# Autodesk Inventor assembly: mezzanineBoard2
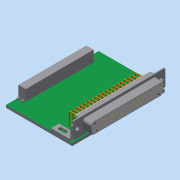
[picture p0: Inventor's stored thumbnail of the model, 180x180]
Saved by Autodesk Inventor 2016 (Build 200138000, 138)
## iProperties
Created: 2016-08-31
Part Number: mezzanineBoard2
Document SubType Name: Assembly
Designer: Zara
Author: Zara
## Documents named in this file (5)
- C:\Users\Zara\Documents\hera-cad\Node\SNAP V2 enclosure release - pack-n-go export\SNAP V2 enclosure release - pack-n-go export\Workspaces\Workspace\components\mezzanineBoard2.iam
- C:\Users\Zara\Documents\hera-cad\Node\SNAP V2 enclosure release - pack-n-go export\SNAP V2 enclosure release - pack-n-go export\Workspaces\Workspace\components\mezzaninePCB.ipt
- C:\Users\Zara\Documents\hera-cad\Node\SNAP V2 enclosure release - pack-n-go export\SNAP V2 enclosure release - pack-n-go export\Workspaces\Workspace\components\snapPinout.ipt
- C:\Users\Zara\Documents\hera-cad\Node\SNAP V2 enclosure release - pack-n-go export\SNAP V2 enclosure release - pack-n-go export\Workspaces\Workspace\components\dsub37Bracket.ipt
- C:\Users\Zara\Documents\hera-cad\Node\SNAP V2 enclosure release - pack-n-go export\SNAP V2 enclosure release - pack-n-go export\Workspaces\Workspace\components\174E-037-213.ipt
## Components (5 placed, 4 different names)
1. mezzaninePCB:1 — Mate:2, Flush:3, Flush:4, Mate:5, Mate:8, Flush:6, Flush:9, Flush:10
2. snapPinout:1 — Mate:2, Flush:3, Flush:4
3. dsub37Bracket:1 — Mate:5, Flush:9, Mate:9
4. dsub37Bracket:2 — Mate:8, Flush:6, Mate:10, Mate:11
5. 174E-037-213:1 — Mate:9, Mate:10, Flush:10, Mate:11
## Relationships (11: Mate 6, Flush 5)
- Mate:2: mezzaninePCB:1 ↔ snapPinout:1
- Flush:3: mezzaninePCB:1 ↔ snapPinout:1
- Flush:4 (9.3 mm): mezzaninePCB:1 ↔ snapPinout:1
- Mate:5: mezzaninePCB:1 ↔ dsub37Bracket:1
- Mate:8: mezzaninePCB:1 ↔ dsub37Bracket:2
- Flush:6: mezzaninePCB:1 ↔ dsub37Bracket:2
- Flush:9: mezzaninePCB:1 ↔ dsub37Bracket:1
- Mate:9: dsub37Bracket:1 ↔ 174E-037-213:1
- Mate:10: dsub37Bracket:2 ↔ 174E-037-213:1
- Flush:10 (0.3277 mm): mezzaninePCB:1 ↔ 174E-037-213:1
- Mate:11: dsub37Bracket:2 ↔ 174E-037-213:1
